# Autodesk Inventor assembly: Main assembly
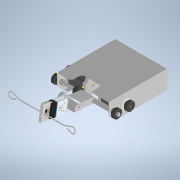
[picture p0: Inventor's stored thumbnail of the model, 180x180]
Saved by Autodesk Inventor 2021 (Build 250183000, 183)
## iProperties
Created: 2020-10-30
Part Number: Main assembly
Document SubType Name: Assembly
Designer: Alfred Brauner
Author: Alfred Brauner
## Documents named in this file (10)
- C:\Users\soeren\Downloads\STOMPA\STOMPA\Main assembly.iam
- C:\Users\soeren\Downloads\STOMPA\STOMPA\RobotChassis.ipt
- C:\Users\soeren\Downloads\STOMPA\STOMPA\Stepper motor NEMA 23HS7430.ipt
- C:\Users\soeren\Downloads\STOMPA\STOMPA\RobotChassis_joint0_Bush.ipt
- C:\Users\soeren\Downloads\STOMPA\STOMPA\Joint0_LongShaft.ipt
- C:\Users\soeren\Downloads\STOMPA\STOMPA\Joint0_Joint1_Bushing.ipt
- C:\Users\soeren\Downloads\STOMPA\STOMPA\Arm Assembly.iam
- C:\Users\soeren\Downloads\STOMPA\STOMPA\Remskive.ipt
- C:\Users\soeren\Downloads\STOMPA\STOMPA\Remskive to huller.ipt
- C:\Users\soeren\Documents\Inventor\Content Center Files\R2021\en-US\BS 3673(2)\BS 3673_1 - B010M.ipt
## Components (17 placed, 9 different names)
1. Frame back plate:1 — Mate:1, Mate:2, Mate:4, Mate:5, Mate:6, Mate:9, Flush:3, Mate:18, Mate:23
2. Stepper motor NEMA 23HS7430:1 — Mate:1, Mate:2, Mate:22, Mate:23, Flush:7
3. Stepper motor NEMA 23HS7430:2 — Mate:4, Mate:5, Mate:6, Mate:24, Flush:8
4. Bos 10:1 — Mate:9, Flush:3, Mate:13
5. Long shaft2:1 — Mate:13, Mate:14, Mate:20, Mate:21
6. BS 3673 : Part 1 - Metric B010M:2
7. BS 3673 : Part 1 - Metric B010M:3
8. Shaft bushing lon o14:1 — Mate:14, Mate:17, Mate:19
9. Arm Assembly:1 [sub-assembly] — Mate:17, Mate:18, Mate:26, Mate:27, Mate:28
10. BS 3673 : Part 1 - Metric B010M:4
11. BS 3673 : Part 1 - Metric B010M:5
12. Remskive:1 — Mate:19
13. Remskive:2 — Mate:20, Flush:9
14. Remskive:3 — Mate:21
15. Remskive:4 — Mate:22, Flush:7
16. Remskive:6 — Mate:24, Flush:8
17. Remskive to huller:1 — Mate:26, Mate:27, Mate:28, Flush:9
## Relationships (28: Mate 23, Flush 4, Insert 1)
- Mate:1: Frame back plate:1 ↔ Stepper motor NEMA 23HS7430:1
- Mate:2: Frame back plate:1 ↔ Stepper motor NEMA 23HS7430:1
- Mate:4: Frame back plate:1 ↔ Stepper motor NEMA 23HS7430:2
- Mate:5: Frame back plate:1 ↔ Stepper motor NEMA 23HS7430:2
- Mate:6: Frame back plate:1 ↔ Stepper motor NEMA 23HS7430:2
- Mate:9: Frame back plate:1 ↔ Bos 10:1
- Flush:3 (2 mm): Frame back plate:1 ↔ Bos 10:1
- [Insert]: Long shaft2:1 ↔ BS 3673 : Part 1 - Metric B010M:2
- [Mate]: Long shaft2:1 ↔ BS 3673 : Part 1 - Metric B010M:3
- [Mate]: Long shaft2:1 ↔ BS 3673 : Part 1 - Metric B010M:3
- Mate:13: Bos 10:1 ↔ Long shaft2:1
- Mate:14: Long shaft2:1 ↔ Shaft bushing lon o14:1
- [Mate]: Long shaft2:1 ↔ BS 3673 : Part 1 - Metric B010M:4
- [Mate]: Long shaft2:1 ↔ BS 3673 : Part 1 - Metric B010M:5
- Mate:17: Shaft bushing lon o14:1 ↔ Arm Assembly:1
- Mate:18 (74.5 mm): Frame back plate:1 ↔ Arm Assembly:1
- Mate:19: Shaft bushing lon o14:1 ↔ Remskive:1
- Mate:20: Long shaft2:1 ↔ Remskive:2
- Mate:21: Long shaft2:1 ↔ Remskive:3
- Mate:22: Stepper motor NEMA 23HS7430:1 ↔ Remskive:4
- Mate:23: Frame back plate:1 ↔ Stepper motor NEMA 23HS7430:1
- Flush:7: Stepper motor NEMA 23HS7430:1 ↔ Remskive:4
- Mate:24: Stepper motor NEMA 23HS7430:2 ↔ Remskive:6
- Flush:8: Stepper motor NEMA 23HS7430:2 ↔ Remskive:6
- Mate:26: Arm Assembly:1 ↔ Remskive to huller:1
- Mate:27: Arm Assembly:1 ↔ Remskive to huller:1
- Mate:28: Arm Assembly:1 ↔ Remskive to huller:1
- Flush:9: Remskive:2 ↔ Remskive to huller:1
